# Autodesk Inventor assembly: звезда и втулка_MIR_MIR1
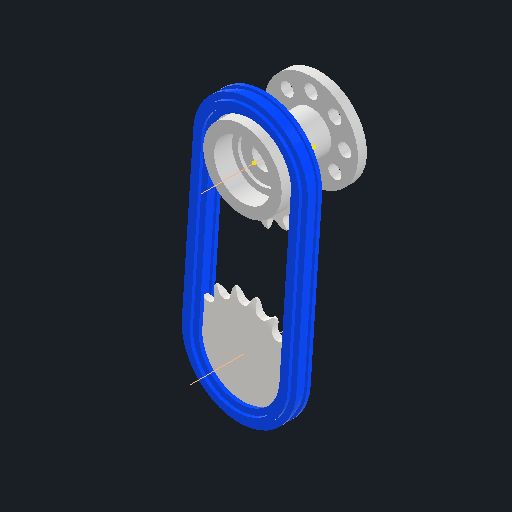
[picture p0: Inventor's stored thumbnail of the model, 512x512]
Saved by Autodesk Inventor 2025 (Build 290162000, 162)
## iProperties
Created: 2024-09-17
Part Number: звезда и втулка_MIR_MIR1
Document SubType Name: Assembly
Designer: GameHD
Author: GameHD
## Documents named in this file (3)
- C:\Users\Phantom\Desktop\Phantom16950\звезда и втулка_MIR_MIR1.iam
- C:\Users\Phantom\Desktop\Phantom16950\втулка для подш_MIR2_MIR.ipt
- C:\Users\Phantom\Desktop\Phantom16950\цепь короткая 2.0_MIR1_MIR.ipt
## Components (2 placed, 2 different names)
1. втулка для подш_MIR2_MIR:1 — Совмещение:1, Заподлицо:1
2. цепь короткая 2.0_MIR1_MIR:1 — Совмещение:1, Заподлицо:1
## Relationships (2: Mate 1, Flush 1)
- Совмещение:1 [Mate]: втулка для подш_MIR2_MIR:1 ↔ цепь короткая 2.0_MIR1_MIR:1
- Заподлицо:1 [Flush] (4 mm): втулка для подш_MIR2_MIR:1 ↔ цепь короткая 2.0_MIR1_MIR:1
